# Autodesk Inventor assembly: newlidassembly
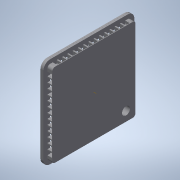
[picture p0: Inventor's stored thumbnail of the model, 180x180]
Saved by Autodesk Inventor 2020 (Build 240168000, 168)
## iProperties
Created: 2019-12-01
Part Number: newlidassembly
Document SubType Name: Assembly
Designer: DDeGo
Author: DDeGo
## Documents named in this file (8)
- C:\Users\DDeGo\Documents\Drew\Projects\LIT pc case\newlidassembly.iam
- C:\Users\DDeGo\Documents\Drew\Projects\LIT pc case\NewFront_A.ipt
- C:\Users\DDeGo\Documents\Drew\Projects\LIT pc case\NewFront_B.ipt
- C:\Users\DDeGo\Documents\Drew\Projects\LIT pc case\NewFront_C.ipt
- C:\Users\DDeGo\Documents\Drew\Projects\LIT pc case\NewFront_D.ipt
- C:\Users\DDeGo\Documents\Drew\Projects\LIT pc case\NewFront_E.ipt
- C:\Users\DDeGo\Documents\Drew\Projects\LIT pc case\NewFront_G.ipt
- C:\Users\DDeGo\Documents\Drew\Projects\LIT pc case\NewFront_H.ipt
## Components (8 placed, 7 different names)
1. NewFront_A:1 — Mate:2, Mate:18, Flush:1, Flush:2, Mate:21, Angle:1
2. NewFront_B:1 — Mate:2, Mate:4, Mate:5, Mate:6, Mate:8, Mate:9, Mate:20, Mate:22, Flush:3
3. NewFront_C:1 — Mate:4, Mate:5, Mate:6, Mate:7
4. NewFront_D:1 — Mate:7, Mate:8, Mate:9, Mate:13, Mate:16, Mate:19
5. NewFront_E:1 — Mate:10, Mate:14, Mate:15
6. NewFront_H:1 — Mate:10, Mate:13, Mate:14, Mate:15, Mate:16, Mate:19
7. NewFront_G:1 — Mate:18, Flush:1, Flush:2
8. NewFront_B:2 — Mate:20, Mate:21, Mate:22, Flush:3, Angle:1
## Relationships (21: Mate 17, Flush 3, Angle 1)
- Mate:2: NewFront_A:1 ↔ NewFront_B:1
- Mate:4: NewFront_B:1 ↔ NewFront_C:1
- Mate:5: NewFront_B:1 ↔ NewFront_C:1
- Mate:6: NewFront_B:1 ↔ NewFront_C:1
- Mate:7: NewFront_C:1 ↔ NewFront_D:1
- Mate:8: NewFront_B:1 ↔ NewFront_D:1
- Mate:9: NewFront_B:1 ↔ NewFront_D:1
- Mate:10: NewFront_E:1 ↔ NewFront_H:1
- Mate:13: NewFront_D:1 ↔ NewFront_H:1
- Mate:14: NewFront_E:1 ↔ NewFront_H:1
- Mate:15: NewFront_E:1 ↔ NewFront_H:1
- Mate:16: NewFront_D:1 ↔ NewFront_H:1
- Mate:18: NewFront_A:1 ↔ NewFront_G:1
- Flush:1: NewFront_A:1 ↔ NewFront_G:1
- Flush:2: NewFront_A:1 ↔ NewFront_G:1
- Mate:19: NewFront_D:1 ↔ NewFront_H:1
- Mate:20: NewFront_B:1 ↔ NewFront_B:2
- Mate:21: NewFront_A:1 ↔ NewFront_B:2
- Mate:22: NewFront_B:1 ↔ NewFront_B:2
- Flush:3: NewFront_B:1 ↔ NewFront_B:2
- Angle:1 (0 deg): NewFront_A:1 ↔ NewFront_B:2
